# Autodesk Inventor assembly: полигон етз
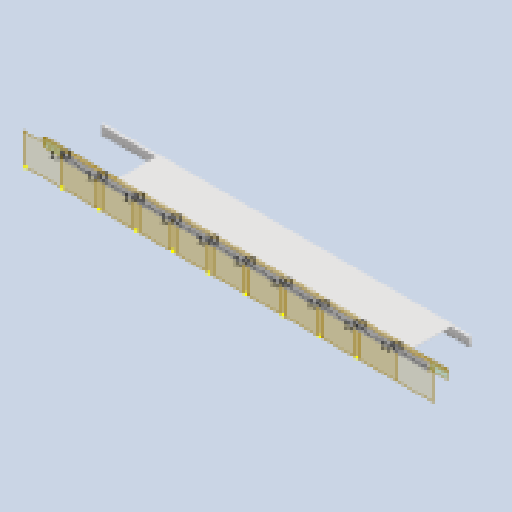
[picture p0: Inventor's stored thumbnail of the model, 512x512]
Saved by Autodesk Inventor 2024.2 (Build 282272000, 272)
## iProperties
Created: 2025-11-16
Part Number: полигон етз
Document SubType Name: Assembly
Designer: katya_notebook
Author: katya_notebook
## Documents named in this file (8)
- C:\Users\91125\OneDrive\Рабочий стол\alletz\полигон етз.iam
- C:\Users\91125\OneDrive\Рабочий стол\alletz\пол.ipt
- C:\Users\91125\Downloads\toothed_rack\m2_20\m2_20.ipt
- C:\Users\91125\Downloads\toothed_rack\m2_20\m2_20_CPY.ipt
- C:\Users\91125\Downloads\toothed_rack\m2_20\m2_20_MIR.ipt
- C:\Users\91125\OneDrive\Документы\брусок.ipt
- C:\Users\91125\OneDrive\Документы\пол2.ipt
- C:\Users\91125\OneDrive\Рабочий стол\alletz\полигон етз_MIR.iam
## Components (35 placed, 7 different names)
1. пол:1
2. m2_20:1 — Совмещение:1, Совмещение:3, Совмещение:4
3. m2_20:2 — Совмещение:1, Совмещение:2, Совмещение:3, Совмещение:4, Совмещение:5, Совмещение:6
4. m2_20:3 — Совмещение:2, Совмещение:5, Совмещение:6, Совмещение:7, Совмещение:8
5. m2_20:4 — Совмещение:7, Совмещение:8, Совмещение:9, Совмещение:10
6. m2_20:5 — Совмещение:9, Совмещение:10, Совмещение:11, Совмещение:12
7. m2_20:6 — Совмещение:15, Совмещение:16, Совмещение:17, Совмещение:18
8. m2_20:7 — Совмещение:17, Совмещение:18, Совмещение:19, Совмещение:20
9. m2_20:8 — Совмещение:11, Совмещение:12, Совмещение:13, Совмещение:14
10. m2_20:9 — Совмещение:19, Совмещение:20
11. m2_20:10 — Совмещение:13, Совмещение:14, Совмещение:15, Совмещение:16
12. m2_20_CPY:1 — Совмещение:21, Совмещение:22, Совмещение:23
13. m2_20_CPY:2 — Совмещение:21, Совмещение:22, Совмещение:23, Совмещение:24, Совмещение:25, Совмещение:26
14. m2_20_CPY:3 — Совмещение:24, Совмещение:25, Совмещение:26, Совмещение:27, Совмещение:28
15. m2_20_CPY:4 — Совмещение:27, Совмещение:28, Совмещение:29, Совмещение:30
16. m2_20_CPY:5 — Совмещение:29, Совмещение:30, Совмещение:33, Совмещение:34
17. m2_20_CPY:6 — Совмещение:31, Совмещение:32, Совмещение:37, Совмещение:38
18. m2_20_CPY:7 — Совмещение:31, Совмещение:32, Совмещение:35, Совмещение:36
19. m2_20_CPY:8 — Совмещение:33, Совмещение:34, Совмещение:39, Совмещение:40
20. m2_20_CPY:9 — Совмещение:35, Совмещение:36
21. m2_20_CPY:10 — Совмещение:37, Совмещение:38, Совмещение:39, Совмещение:40
22. m2_20_MIR:1 — Совмещение:44, Совмещение:45, Совмещение:46
23. m2_20_MIR:2 — Совмещение:44, Совмещение:45, Совмещение:46, Совмещение:47, Совмещение:48, Совмещение:49
24. m2_20_MIR:3 — Совмещение:47, Совмещение:48, Совмещение:49, Совмещение:50, Совмещение:51
25. m2_20_MIR:4 — Совмещение:50, Совмещение:51, Совмещение:52, Совмещение:53
26. m2_20_MIR:5 — Совмещение:52, Совмещение:53, Совмещение:56, Совмещение:57
27. m2_20_MIR:6 — Совмещение:54, Совмещение:55, Совмещение:60, Совмещение:61
28. m2_20_MIR:7 — Совмещение:54, Совмещение:55, Совмещение:58, Совмещение:59
29. m2_20_MIR:8 — Совмещение:56, Совмещение:57, Совмещение:62, Совмещение:63
30. m2_20_MIR:9 — Совмещение:58, Совмещение:59, Заподлицо:5, Совмещение:67
31. полигон етз_MIR:1 [sub-assembly] — Совмещение:66
32. m2_20_MIR:10 — Совмещение:60, Совмещение:61, Совмещение:62, Совмещение:63
33. брусок:1 — Заподлицо:5, Заподлицо:8, Совмещение:66, Совмещение:67, Заподлицо:9
34. пол:2 — Совмещение:68
35. пол2:1 — Заподлицо:8, Совмещение:68
## Relationships (68: Mate 65, Flush 3)
- Совмещение:1 [Mate]: m2_20:1 ↔ m2_20:2
- Совмещение:2 [Mate]: m2_20:2 ↔ m2_20:3
- Совмещение:3 [Mate]: m2_20:1 ↔ m2_20:2
- Совмещение:4 [Mate]: m2_20:1 ↔ m2_20:2
- Совмещение:5 [Mate]: m2_20:2 ↔ m2_20:3
- Совмещение:6 [Mate]: m2_20:2 ↔ m2_20:3
- Совмещение:7 [Mate]: m2_20:3 ↔ m2_20:4
- Совмещение:8 [Mate]: m2_20:3 ↔ m2_20:4
- Совмещение:9 [Mate]: m2_20:4 ↔ m2_20:5
- Совмещение:10 [Mate]: m2_20:4 ↔ m2_20:5
- Совмещение:11 [Mate]: m2_20:5 ↔ m2_20:8
- Совмещение:12 [Mate]: m2_20:5 ↔ m2_20:8
- Совмещение:13 [Mate]: m2_20:8 ↔ m2_20:10
- Совмещение:14 [Mate]: m2_20:8 ↔ m2_20:10
- Совмещение:15 [Mate]: m2_20:6 ↔ m2_20:10
- Совмещение:16 [Mate]: m2_20:6 ↔ m2_20:10
- Совмещение:17 [Mate]: m2_20:6 ↔ m2_20:7
- Совмещение:18 [Mate]: m2_20:6 ↔ m2_20:7
- Совмещение:19 [Mate]: m2_20:7 ↔ m2_20:9
- Совмещение:20 [Mate]: m2_20:7 ↔ m2_20:9
- Совмещение:21 [Mate]: m2_20_CPY:1 ↔ m2_20_CPY:2
- Совмещение:22 [Mate]: m2_20_CPY:1 ↔ m2_20_CPY:2
- Совмещение:23 [Mate]: m2_20_CPY:1 ↔ m2_20_CPY:2
- Совмещение:24 [Mate]: m2_20_CPY:2 ↔ m2_20_CPY:3
- Совмещение:25 [Mate]: m2_20_CPY:2 ↔ m2_20_CPY:3
- Совмещение:26 [Mate]: m2_20_CPY:2 ↔ m2_20_CPY:3
- Совмещение:27 [Mate]: m2_20_CPY:3 ↔ m2_20_CPY:4
- Совмещение:28 [Mate]: m2_20_CPY:3 ↔ m2_20_CPY:4
- Совмещение:29 [Mate]: m2_20_CPY:4 ↔ m2_20_CPY:5
- Совмещение:30 [Mate]: m2_20_CPY:4 ↔ m2_20_CPY:5
- Совмещение:31 [Mate]: m2_20_CPY:6 ↔ m2_20_CPY:7
- Совмещение:32 [Mate]: m2_20_CPY:6 ↔ m2_20_CPY:7
- Совмещение:33 [Mate]: m2_20_CPY:5 ↔ m2_20_CPY:8
- Совмещение:34 [Mate]: m2_20_CPY:5 ↔ m2_20_CPY:8
- Совмещение:35 [Mate]: m2_20_CPY:7 ↔ m2_20_CPY:9
- Совмещение:36 [Mate]: m2_20_CPY:7 ↔ m2_20_CPY:9
- Совмещение:37 [Mate]: m2_20_CPY:6 ↔ m2_20_CPY:10
- Совмещение:38 [Mate]: m2_20_CPY:6 ↔ m2_20_CPY:10
- Совмещение:39 [Mate]: m2_20_CPY:8 ↔ m2_20_CPY:10
- Совмещение:40 [Mate]: m2_20_CPY:8 ↔ m2_20_CPY:10
- Совмещение:44 [Mate]: m2_20_MIR:1 ↔ m2_20_MIR:2
- Совмещение:45 [Mate]: m2_20_MIR:1 ↔ m2_20_MIR:2
- Совмещение:46 [Mate]: m2_20_MIR:1 ↔ m2_20_MIR:2
- Совмещение:47 [Mate]: m2_20_MIR:2 ↔ m2_20_MIR:3
- Совмещение:48 [Mate]: m2_20_MIR:2 ↔ m2_20_MIR:3
- Совмещение:49 [Mate]: m2_20_MIR:2 ↔ m2_20_MIR:3
- Совмещение:50 [Mate]: m2_20_MIR:3 ↔ m2_20_MIR:4
- Совмещение:51 [Mate]: m2_20_MIR:3 ↔ m2_20_MIR:4
- Совмещение:52 [Mate]: m2_20_MIR:4 ↔ m2_20_MIR:5
- Совмещение:53 [Mate]: m2_20_MIR:4 ↔ m2_20_MIR:5
- Совмещение:54 [Mate]: m2_20_MIR:6 ↔ m2_20_MIR:7
- Совмещение:55 [Mate]: m2_20_MIR:6 ↔ m2_20_MIR:7
- Совмещение:56 [Mate]: m2_20_MIR:5 ↔ m2_20_MIR:8
- Совмещение:57 [Mate]: m2_20_MIR:5 ↔ m2_20_MIR:8
- Совмещение:58 [Mate]: m2_20_MIR:7 ↔ m2_20_MIR:9
- Совмещение:59 [Mate]: m2_20_MIR:7 ↔ m2_20_MIR:9
- Совмещение:60 [Mate]: m2_20_MIR:6 ↔ m2_20_MIR:10
- Совмещение:61 [Mate]: m2_20_MIR:6 ↔ m2_20_MIR:10
- Совмещение:62 [Mate]: m2_20_MIR:8 ↔ m2_20_MIR:10
- Совмещение:63 [Mate]: m2_20_MIR:8 ↔ m2_20_MIR:10
- Заподлицо:5 [Flush]: m2_20_MIR:9 ↔ брусок:1
- Заподлицо:8 [Flush]: брусок:1 ↔ пол2:1
- [Mate]: полигон етз_MIR:1 ↔ брусок:1
- [Mate]: полигон етз_MIR:1 ↔ брусок:1
- Совмещение:66 [Mate]: полигон етз_MIR:1 ↔ брусок:1
- Совмещение:67 [Mate]: m2_20_MIR:9 ↔ брусок:1
- Совмещение:68 [Mate]: пол:2 ↔ пол2:1
- Заподлицо:9 [Flush] (-8 mm): брусок:1
## Named parameters: d72_d5 = 0 mm, d73_d6 = 0 mm
